# Autodesk Inventor assembly: SNAP 8x10x1 Ver1.A
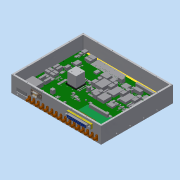
[picture p0: Inventor's stored thumbnail of the model, 180x180]
Saved by Autodesk Inventor 2016 (Build 200138000, 138)
## iProperties
Created: 2015-07-14
Part Number: SNAP 8x10x1 Ver1.A
Document SubType Name: Assembly
Designer: rtreacy
Author: rtreacy
## Documents named in this file (18)
- C:\Users\Zara\Documents\hera-cad\Node\SNAP V2 enclosure release - pack-n-go export\SNAP V2 enclosure release - pack-n-go export\Workspaces\Workspace\SNAP 8x10x1.75 Ver1.A.iam
- C:\Users\Zara\Documents\hera-cad\Node\SNAP V2 enclosure release - pack-n-go export\SNAP V2 enclosure release - pack-n-go export\Workspaces\Workspace\components\R58010-175-with SNAP V2 features.ipt
- C:\Users\Zara\Documents\hera-cad\Node\SNAP V2 enclosure release - pack-n-go export\SNAP V2 enclosure release - pack-n-go export\Workspaces\Workspace\components\mounting rail 7.0 x.250 x .250.ipt
- C:\Users\Zara\Documents\hera-cad\Node\SNAP V2 enclosure release - pack-n-go export\SNAP V2 enclosure release - pack-n-go export\Workspaces\Workspace\components\mounting rail 9.0 x.250 x.500-A.ipt
- C:\Users\Zara\Documents\hera-cad\Node\SNAP V2 enclosure release - pack-n-go export\SNAP V2 enclosure release - pack-n-go export\Workspaces\Workspace\components\mounting rail 9.0 x.250 x.500-B.ipt
- C:\Users\Zara\Documents\hera-cad\Node\SNAP V2 enclosure release - pack-n-go export\SNAP V2 enclosure release - pack-n-go export\Workspaces\Workspace\imports\132143_iges_file.ipt
- C:\Users\Zara\Documents\hera-cad\Node\SNAP V2 enclosure release - pack-n-go export\SNAP V2 enclosure release - pack-n-go export\Workspaces\Workspace\components\RFT 8x10 Cover Ext.ipt
- C:\Users\Zara\Documents\hera-cad\Node\SNAP V2 enclosure release - pack-n-go export\SNAP V2 enclosure release - pack-n-go export\Workspaces\Workspace\components\RFT 8x10 Cover.ipt
- C:\Users\Zara\Documents\hera-cad\Node\SNAP V2 enclosure release - pack-n-go export\SNAP V2 enclosure release - pack-n-go export\Workspaces\Workspace\drawings\SNAP Ver2 pack-n-go\Workgroups\NotInProject\SNAP-V2_1_0.iam
- C:\Users\Zara\Documents\hera-cad\Node\SNAP V2 enclosure release - pack-n-go export\SNAP V2 enclosure release - pack-n-go export\Workspaces\Workspace\components\Top Heat Sink.ipt
- C:\Users\Zara\Documents\hera-cad\Node\SNAP V2 enclosure release - pack-n-go export\SNAP V2 enclosure release - pack-n-go export\Workspaces\Workspace\components\Thermal pad .100.ipt
- C:\Users\Zara\Documents\hera-cad\Node\SNAP V2 enclosure release - pack-n-go export\SNAP V2 enclosure release - pack-n-go export\Workspaces\Workspace\components\Bot Heat Sink.ipt
- C:\Users\Zara\Documents\hera-cad\Node\SNAP V2 enclosure release - pack-n-go export\SNAP V2 enclosure release - pack-n-go export\Workspaces\Workspace\components\RFT 8x10 Cover-alt-base.ipt
- C:\Users\Zara\Documents\hera-cad\Node\SNAP V2 enclosure release - pack-n-go export\SNAP V2 enclosure release - pack-n-go export\Workspaces\Workspace\components\mezzanineBoard.iam
- C:\Users\Zara\Documents\hera-cad\Node\SNAP V2 enclosure release - pack-n-go export\SNAP V2 enclosure release - pack-n-go export\Workspaces\Workspace\components\c-5747024-3-a-3d.ipt
- C:\Users\Zara\Documents\hera-cad\Node\SNAP V2 enclosure release - pack-n-go export\SNAP V2 enclosure release - pack-n-go export\Workspaces\Workspace\components\GCLP37M37F.iam
- C:\Users\Zara\Documents\hera-cad\Node\SNAP V2 enclosure release - pack-n-go export\SNAP V2 enclosure release - pack-n-go export\Workspaces\Workspace\components\dsub9API.iam
- C:\Users\Zara\Documents\hera-cad\Node\SNAP V2 enclosure release - pack-n-go export\SNAP V2 enclosure release - pack-n-go export\Workspaces\Workspace\components\ENG_CVM_CVM_745777-4_D.3d_stp\c-745777-4-d-3d.ipt
## Components (34 placed, 17 different names)
1. R58010-175-with SNAP V2 features:1 — Mate:1, Mate:2, Insert:1, Insert:2, Insert:3, Insert:4, Insert:5, Insert:6, Insert:7, Insert:8, Insert:9, Insert:10, Insert:11, Insert:12, Insert:13, Insert:14, Insert:15, Insert:16, Mate:8, Mate:9, Mate:10, Mate:11, Mate:13, Angle:1, Angle:2, Angle:3, Angle:4, Angle:5, Angle:6, Angle:7, Angle:8, Angle:9, Angle:10, Angle:11, Angle:12, Angle:13, Angle:14, Angle:15, Angle:16, Mate:17, Flush:3, Flush:4, Mate:20, Flush:5, Mate:21, Mate:35, Mate:36, Mate:37, Mate:46, Mate:55, Mate:56, Mate:57, Mate:58, Mate:59, Mate:61, Mate:62, Mate:63, Mate:64, Mate:65, Mate:66, Mate:67, Mate:68
2. mounting rail 7.0 x.250 x .250:1 — Mate:1, Flush:1, Mate:11, Mate:16
3. mounting rail 7.0 x.250 x .250:2 — Mate:2, Flush:2, Mate:8
4. mounting rail 9.0 x.250 x.500-A:1 — Flush:2, Mate:10, Mate:13, Mate:14
5. mounting rail 9.0 x.250 x.500-B:1 — Flush:1, Mate:9
6. 132143_iges_file:1 — Insert:1, Angle:1
7. 132143_iges_file:2 — Insert:2, Angle:2
8. 132143_iges_file:3 — Insert:3, Angle:3
9. 132143_iges_file:4 — Insert:4, Angle:4
10. 132143_iges_file:5 — Insert:5, Angle:5
11. 132143_iges_file:6 — Insert:6, Angle:6
12. 132143_iges_file:7 — Insert:7, Angle:7
13. 132143_iges_file:8 — Insert:8, Angle:8
14. 132143_iges_file:9 — Insert:9, Angle:9
15. 132143_iges_file:10 — Insert:10, Angle:10
16. 132143_iges_file:11 — Insert:11, Angle:11
17. 132143_iges_file:12 — Insert:12, Angle:12
18. 132143_iges_file:13 — Insert:13, Angle:13
19. 132143_iges_file:14 — Insert:14, Angle:14
20. 132143_iges_file:15 — Insert:15, Angle:15
21. 132143_iges_file:16 — Insert:16, Angle:16
22. RFT 8x10 Cover Ext:1 — Mate:20, Flush:5, Mate:21, Mate:32, Mate:33, Mate:34
23. RFT 8x10 Cover:1 — Mate:17, Flush:3, Flush:4, Mate:27, Mate:28, Mate:29, Mate:30
24. SNAP-V2_1_0:1 [sub-assembly] — Mate:14, Mate:16
25. Top Heat Sink:1 — Mate:24, Mate:25, Flush:6, Flush:7, Mate:27, Mate:28, Mate:29, Mate:30
26. Thermal pad .100:1 — Mate:24, Mate:25, Flush:6, Flush:7
27. Thermal pad .100:2 — Mate:31, Flush:8, Flush:9
28. Bot Heat Sink:1 — Mate:31, Flush:8, Flush:9, Mate:32, Mate:33, Mate:34
29. RFT 8x10 Cover-alt-base:1 — Mate:35, Mate:36, Mate:37
30. mezzanineBoard:1 [sub-assembly] — Mate:58, Mate:59, Mate:60
31. c-5747024-3-a-3d:1 — Mate:46, Mate:64, Mate:65, Mate:66, Mate:69
32. GCLP37M37F:1 [sub-assembly] — Mate:61, Mate:62, Mate:63
33. dsub9API:1 [sub-assembly] — Mate:67, Mate:68, Mate:69
34. c-745777-4-d-3d:1 — Mate:55, Mate:56, Mate:57, Mate:60
## Relationships (82: Mate 41, Insert 16, Angle 16, Flush 9)
- Mate:1: R58010-175-with SNAP V2 features:1 ↔ mounting rail 7.0 x.250 x .250:1
- Mate:2: R58010-175-with SNAP V2 features:1 ↔ mounting rail 7.0 x.250 x .250:2
- Insert:1: R58010-175-with SNAP V2 features:1 ↔ 132143_iges_file:1
- Insert:2: R58010-175-with SNAP V2 features:1 ↔ 132143_iges_file:2
- Insert:3: R58010-175-with SNAP V2 features:1 ↔ 132143_iges_file:3
- Insert:4: R58010-175-with SNAP V2 features:1 ↔ 132143_iges_file:4
- Insert:5: R58010-175-with SNAP V2 features:1 ↔ 132143_iges_file:5
- Insert:6: R58010-175-with SNAP V2 features:1 ↔ 132143_iges_file:6
- Insert:7: R58010-175-with SNAP V2 features:1 ↔ 132143_iges_file:7
- Insert:8: R58010-175-with SNAP V2 features:1 ↔ 132143_iges_file:8
- Insert:9: R58010-175-with SNAP V2 features:1 ↔ 132143_iges_file:9
- Insert:10: R58010-175-with SNAP V2 features:1 ↔ 132143_iges_file:10
- Insert:11: R58010-175-with SNAP V2 features:1 ↔ 132143_iges_file:11
- Insert:12: R58010-175-with SNAP V2 features:1 ↔ 132143_iges_file:12
- Insert:13: R58010-175-with SNAP V2 features:1 ↔ 132143_iges_file:13
- Insert:14: R58010-175-with SNAP V2 features:1 ↔ 132143_iges_file:14
- Insert:15: R58010-175-with SNAP V2 features:1 ↔ 132143_iges_file:15
- Insert:16: R58010-175-with SNAP V2 features:1 ↔ 132143_iges_file:16
- Flush:1: mounting rail 7.0 x.250 x .250:1 ↔ mounting rail 9.0 x.250 x.500-B:1
- Flush:2: mounting rail 7.0 x.250 x .250:2 ↔ mounting rail 9.0 x.250 x.500-A:1
- Mate:8: R58010-175-with SNAP V2 features:1 ↔ mounting rail 7.0 x.250 x .250:2
- Mate:9: R58010-175-with SNAP V2 features:1 ↔ mounting rail 9.0 x.250 x.500-B:1
- Mate:10: R58010-175-with SNAP V2 features:1 ↔ mounting rail 9.0 x.250 x.500-A:1
- Mate:11: R58010-175-with SNAP V2 features:1 ↔ mounting rail 7.0 x.250 x .250:1
- Mate:13: R58010-175-with SNAP V2 features:1 ↔ mounting rail 9.0 x.250 x.500-A:1
- Angle:1 (0 deg): R58010-175-with SNAP V2 features:1 ↔ 132143_iges_file:1
- Angle:2 (0 deg): R58010-175-with SNAP V2 features:1 ↔ 132143_iges_file:2
- Angle:3 (0 deg): R58010-175-with SNAP V2 features:1 ↔ 132143_iges_file:3
- Angle:4 (0 deg): R58010-175-with SNAP V2 features:1 ↔ 132143_iges_file:4
- Angle:5 (0 deg): R58010-175-with SNAP V2 features:1 ↔ 132143_iges_file:5
- Angle:6 (0 deg): R58010-175-with SNAP V2 features:1 ↔ 132143_iges_file:6
- Angle:7 (0 deg): R58010-175-with SNAP V2 features:1 ↔ 132143_iges_file:7
- Angle:8 (0 deg): R58010-175-with SNAP V2 features:1 ↔ 132143_iges_file:8
- Angle:9 (0 deg): R58010-175-with SNAP V2 features:1 ↔ 132143_iges_file:9
- Angle:10 (0 deg): R58010-175-with SNAP V2 features:1 ↔ 132143_iges_file:10
- Angle:11 (0 deg): R58010-175-with SNAP V2 features:1 ↔ 132143_iges_file:11
- Angle:12 (0 deg): R58010-175-with SNAP V2 features:1 ↔ 132143_iges_file:12
- Angle:13 (0 deg): R58010-175-with SNAP V2 features:1 ↔ 132143_iges_file:13
- Angle:14 (0 deg): R58010-175-with SNAP V2 features:1 ↔ 132143_iges_file:14
- Angle:15 (0 deg): R58010-175-with SNAP V2 features:1 ↔ 132143_iges_file:15
- Angle:16 (0 deg): R58010-175-with SNAP V2 features:1 ↔ 132143_iges_file:16
- Mate:14: mounting rail 9.0 x.250 x.500-A:1 ↔ SNAP-V2_1_0:1
- Mate:16: mounting rail 7.0 x.250 x .250:1 ↔ SNAP-V2_1_0:1
- Mate:17: R58010-175-with SNAP V2 features:1 ↔ RFT 8x10 Cover:1
- Flush:3: R58010-175-with SNAP V2 features:1 ↔ RFT 8x10 Cover:1
- Flush:4: R58010-175-with SNAP V2 features:1 ↔ RFT 8x10 Cover:1
- Mate:20: R58010-175-with SNAP V2 features:1 ↔ RFT 8x10 Cover Ext:1
- Flush:5: R58010-175-with SNAP V2 features:1 ↔ RFT 8x10 Cover Ext:1
- Mate:21: R58010-175-with SNAP V2 features:1 ↔ RFT 8x10 Cover Ext:1
- Mate:24: Top Heat Sink:1 ↔ Thermal pad .100:1
- Mate:25: Top Heat Sink:1 ↔ Thermal pad .100:1
- Flush:6: Top Heat Sink:1 ↔ Thermal pad .100:1
- Flush:7: Top Heat Sink:1 ↔ Thermal pad .100:1
- Mate:27: RFT 8x10 Cover:1 ↔ Top Heat Sink:1
- Mate:28: RFT 8x10 Cover:1 ↔ Top Heat Sink:1
- Mate:29: RFT 8x10 Cover:1 ↔ Top Heat Sink:1
- Mate:30: RFT 8x10 Cover:1 ↔ Top Heat Sink:1
- Mate:31: Thermal pad .100:2 ↔ Bot Heat Sink:1
- Flush:8: Thermal pad .100:2 ↔ Bot Heat Sink:1
- Flush:9: Thermal pad .100:2 ↔ Bot Heat Sink:1
- Mate:32: RFT 8x10 Cover Ext:1 ↔ Bot Heat Sink:1
- Mate:33: RFT 8x10 Cover Ext:1 ↔ Bot Heat Sink:1
- Mate:34: RFT 8x10 Cover Ext:1 ↔ Bot Heat Sink:1
- Mate:35: R58010-175-with SNAP V2 features:1 ↔ RFT 8x10 Cover-alt-base:1
- Mate:36: R58010-175-with SNAP V2 features:1 ↔ RFT 8x10 Cover-alt-base:1
- Mate:37: R58010-175-with SNAP V2 features:1 ↔ RFT 8x10 Cover-alt-base:1
- Mate:46: R58010-175-with SNAP V2 features:1 ↔ c-5747024-3-a-3d:1
- Mate:55: R58010-175-with SNAP V2 features:1 ↔ c-745777-4-d-3d:1
- Mate:56: R58010-175-with SNAP V2 features:1 ↔ c-745777-4-d-3d:1
- Mate:57: R58010-175-with SNAP V2 features:1 ↔ c-745777-4-d-3d:1
- Mate:58: R58010-175-with SNAP V2 features:1 ↔ mezzanineBoard:1
- Mate:59: R58010-175-with SNAP V2 features:1 ↔ mezzanineBoard:1
- Mate:60: mezzanineBoard:1 ↔ c-745777-4-d-3d:1
- Mate:61: R58010-175-with SNAP V2 features:1 ↔ GCLP37M37F:1
- Mate:62: R58010-175-with SNAP V2 features:1 ↔ GCLP37M37F:1
- Mate:63: R58010-175-with SNAP V2 features:1 ↔ GCLP37M37F:1
- Mate:64: R58010-175-with SNAP V2 features:1 ↔ c-5747024-3-a-3d:1
- Mate:65: R58010-175-with SNAP V2 features:1 ↔ c-5747024-3-a-3d:1
- Mate:66: R58010-175-with SNAP V2 features:1 ↔ c-5747024-3-a-3d:1
- Mate:67: R58010-175-with SNAP V2 features:1 ↔ dsub9API:1
- Mate:68: R58010-175-with SNAP V2 features:1 ↔ dsub9API:1
- Mate:69: c-5747024-3-a-3d:1 ↔ dsub9API:1
